# Autodesk Inventor assembly: 下半身_6
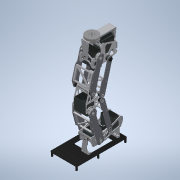
[picture p0: Inventor's stored thumbnail of the model, 180x180]
Saved by Autodesk Inventor 2020 (Build 240168000, 168)
## iProperties
Created: 2016-08-23
Part Number: 下半身_6
Material: 一般
Document SubType Name: Assembly
Designer: hiro
Mass: 967.04 g
Surface Area: 2501.85 cm^2
Volume: 430.712 cm^3
Density: 2.24521 g/cm^3
Author: hiro
## Documents named in this file (14)
- C:\Users\Masato\Documents\Inventor\CIT Brains_Inventor\OpenPlatform_ver3_0\下半身_MIR.iam
- C:\Users\Masato\Documents\Inventor\CIT Brains_Inventor\OpenPlatform_ver3_0\下半身\足首\足首_独立ピッチ_1.iam
- C:\Users\Masato\Documents\Inventor\CIT Brains_Inventor\OpenPlatform_ver3_0\下半身_160823\リンク\リンク_6_2.iam
- C:\Users\Masato\Documents\Inventor\CIT Brains_Inventor\OpenPlatform_ver3_0\下半身_160823\リンク\リンク_6_3.iam
- C:\Users\Masato\Documents\Inventor\CIT Brains_Inventor\OpenPlatform_ver3_0\下半身_160823\リンク\リンク_6_4.iam
- C:\Users\Masato\Documents\Inventor\CIT Brains_Inventor\OpenPlatform_ver3_0\下半身_160823\付け根ロール\付け根ロール_1.iam
- C:\Users\Masato\Documents\Inventor\CIT Brains_Inventor\OpenPlatform_ver3_0\下半身\足裏\足裏_1_1_MIR.iam
- C:\Users\Masato\Documents\Inventor\CIT Brains_Inventor\OpenPlatform_ver3_0\下半身_160823\膝\膝_6_1_MIR.iam
- C:\Users\Masato\Documents\Inventor\CIT Brains_Inventor\OpenPlatform_ver3_0\下半身_160823\リンク\リンク_ふくらはぎ_サブフレーム_1_4.ipt
- C:\Users\Masato\Documents\Inventor\CIT Brains_Inventor\OpenPlatform_ver3_0\下半身\足首\足首_1_MIR.iam
- C:\Users\Masato\Documents\Inventor\CIT Brains_Inventor\OpenPlatform_ver3_0\下半身_160823\リンク\リンク_6_1.iam
- C:\Users\Masato\Documents\Inventor\CIT Brains_Inventor\OpenPlatform_ver3_0\下半身_160823\付け根\付け根_1_MIR2.iam
- C:\Users\Masato\Documents\Inventor\CIT Brains_Inventor\OpenPlatform_ver3_0\既製品\WSSS12-10-6.ipt
- C:\Users\Masato\Documents\Inventor\CIT Brains_Inventor\OpenPlatform_ver3_0\下半身\長穴減速\長穴減速_ホーン.iam
## Components (19 placed, 13 different names)
1. 付け根ロール_1:1 [sub-assembly] — メイト:23, フラッシュ:25, フラッシュ:26, 角度:33, 挿入:118, 挿入:128
2. 足首_独立ピッチ_1:1 [sub-assembly] — 挿入:87, 挿入:100, 挿入:102
3. リンク_6_4:1 [sub-assembly] — 角度:18, 角度:19, 角度:20, 角度:21, 挿入:112, 挿入:121, 挿入:123, 挿入:125
4. リンク_6_2:1 [sub-assembly] — 角度:14, 角度:15, 角度:17, 挿入:87, 角度:32, 挿入:122, 挿入:124, 挿入:126
5. 足裏_1_1_MIR:1 [sub-assembly] — 角度:33, 挿入:101
6. 膝_6_1_MIR:1 [sub-assembly] — 角度:20, 角度:18, 角度:14, 角度:15, 角度:19, 角度:17, 角度:21, 挿入:76, 挿入:77, 挿入:78, 挿入:79, 角度:30, 角度:32, 挿入:112, 挿入:113, 挿入:114
7. リンク_ふくらはぎ_サブフレーム_1_4:1
8. リンク_ふくらはぎ_サブフレーム_1_4:2 — 挿入:119, 挿入:121
9. リンク_ふくらはぎ_サブフレーム_1_4:3 — 挿入:78, 挿入:79
10. リンク_ふくらはぎ_サブフレーム_1_4:4 — 挿入:76, 挿入:77, 挿入:122
11. リンク_6_3:2 [sub-assembly] — 挿入:113, 挿入:117
12. 足首_1_MIR:1 [sub-assembly] — 角度:30, 挿入:101, 挿入:102
13. リンク_6_1:1 [sub-assembly] — 挿入:100, 挿入:114
14. 付け根_1_MIR1:1 [sub-assembly] — 挿入:117, 挿入:118, 挿入:119, 挿入:127
15. WSSS12-10-6:1 — 挿入:123
16. WSSS12-10-6:2 — 挿入:124
17. WSSS12-10-6:3 — 挿入:125
18. WSSS12-10-6:4 — 挿入:126
19. 長穴減速_ホーン:1 [sub-assembly] — 挿入:127, 挿入:128
## Relationships (35: Insert 22, Angle 10, Flush 2, Mate 1)
- 角度:14 [Angle] (0 deg): リンク_6_2:1 ↔ 膝_6_1_MIR:1
- 角度:15 [Angle] (-30 deg): リンク_6_2:1 ↔ 膝_6_1_MIR:1
- 角度:17 [Angle] (90 deg): リンク_6_2:1 ↔ 膝_6_1_MIR:1
- 角度:18 [Angle] (0 deg): リンク_6_4:1 ↔ 膝_6_1_MIR:1
- 角度:19 [Angle] (30 deg): リンク_6_4:1 ↔ 膝_6_1_MIR:1
- 角度:20 [Angle] (15 deg): リンク_6_4:1 ↔ 膝_6_1_MIR:1
- 角度:21 [Angle] (90 deg): リンク_6_4:1 ↔ 膝_6_1_MIR:1
- メイト:23 [Mate]: 付け根ロール_1:1
- フラッシュ:25 [Flush]: 付け根ロール_1:1
- フラッシュ:26 [Flush]: 付け根ロール_1:1
- 挿入:76 [Insert]: 膝_6_1_MIR:1 ↔ リンク_ふくらはぎ_サブフレーム_1_4:4
- 挿入:77 [Insert]: 膝_6_1_MIR:1 ↔ リンク_ふくらはぎ_サブフレーム_1_4:4
- 挿入:78 [Insert]: 膝_6_1_MIR:1 ↔ リンク_ふくらはぎ_サブフレーム_1_4:3
- 挿入:79 [Insert]: 膝_6_1_MIR:1 ↔ リンク_ふくらはぎ_サブフレーム_1_4:3
- 挿入:87 [Insert]: 足首_独立ピッチ_1:1 ↔ リンク_6_2:1
- 角度:30 [Angle] (0 deg): 膝_6_1_MIR:1 ↔ 足首_1_MIR:1
- 角度:32 [Angle] (-15 deg): リンク_6_2:1 ↔ 膝_6_1_MIR:1
- 挿入:100 [Insert]: 足首_独立ピッチ_1:1 ↔ リンク_6_1:1
- 角度:33 [Angle] (180 deg): 付け根ロール_1:1 ↔ 足裏_1_1_MIR:1
- 挿入:101 [Insert]: 足裏_1_1_MIR:1 ↔ 足首_1_MIR:1
- 挿入:102 [Insert]: 足首_独立ピッチ_1:1 ↔ 足首_1_MIR:1
- 挿入:112 [Insert]: リンク_6_4:1 ↔ 膝_6_1_MIR:1
- 挿入:113 [Insert]: 膝_6_1_MIR:1 ↔ リンク_6_3:2
- 挿入:114 [Insert]: 膝_6_1_MIR:1 ↔ リンク_6_1:1
- 挿入:117 [Insert]: リンク_6_3:2 ↔ 付け根_1_MIR1:1
- 挿入:118 [Insert]: 付け根ロール_1:1 ↔ 付け根_1_MIR1:1
- 挿入:119 [Insert]: リンク_ふくらはぎ_サブフレーム_1_4:2 ↔ 付け根_1_MIR1:1
- 挿入:121 [Insert]: リンク_6_4:1 ↔ リンク_ふくらはぎ_サブフレーム_1_4:2
- 挿入:122 [Insert]: リンク_6_2:1 ↔ リンク_ふくらはぎ_サブフレーム_1_4:4
- 挿入:123 [Insert]: リンク_6_4:1 ↔ WSSS12-10-6:1
- 挿入:124 [Insert]: リンク_6_2:1 ↔ WSSS12-10-6:2
- 挿入:125 [Insert]: リンク_6_4:1 ↔ WSSS12-10-6:3
- 挿入:126 [Insert]: リンク_6_2:1 ↔ WSSS12-10-6:4
- 挿入:127 [Insert]: 付け根_1_MIR1:1 ↔ 長穴減速_ホーン:1
- 挿入:128 [Insert]: 付け根ロール_1:1 ↔ 長穴減速_ホーン:1
## Named parameters: sa_0 = 80000, sa_1 = -5.398e-10, sa_2 = 3.965e-10
note: some values were not read from the file. Shown as the stored number, unit unknown: "sa_0", "sa_1", "sa_2".
